# Autodesk Inventor assembly: M178-1000
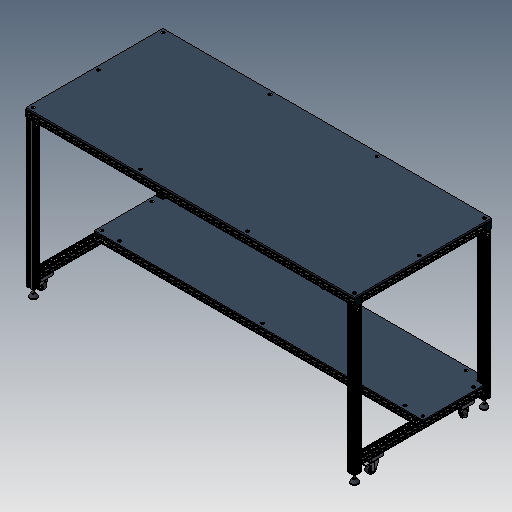
[picture p0: Inventor's stored thumbnail of the model, 512x512]
Saved by Autodesk Inventor 2018.3 (Build 223284000, 284)
## iProperties
Created: 2004-11-17
Part Number: M178-1000
Document SubType Name: Assembly
Designer: Autodesk, Inc.
Manufacturer: Standard
Standards Organization: Custom
Description: TABLE, MAIN
Mass: 47415.2 g
Surface Area: 115729 cm^2
Volume: 28165.1 cm^3
Density: 1.68347 g/cm^3
CAGE: 1LJX3
Dept. ID: Product Design
Description #2: ---
Finish #1: ---
Finish #2: ---
Material ID: ---
Project Number: ---
Author: Autodesk, Inc.
## Documents named in this file (14)
- C:\AVAInvAPI\Workspace\Test Station\Components\M178-1000.iam
- C:\AVAInvAPI\Workspace\Test Station\Components\M178-1001.ipt
- C:\AVAInvAPI\Workspace\Test Station\Components\M178-1007.ipt
- C:\AVAInvAPI\Workspace\Test Station\Components\M178-1005.ipt
- C:\AVAInvAPI\Workspace\Test Station\Components\M178-1100.iam
- C:\AVAInvAPI\Workspace\Test Station\Components\M178-1000-Phantom01.iam
- C:\AVAInvAPI\Workspace\Test Station\Components\M178-1000_Leg_Phantom.iam
- C:\AVAInvAPI\Workspace\Test Station\Components\18-813.ipt
- C:\AVAInvAPI\Workspace\Test Station\Components\20-004.iam
- C:\AVAInvAPI\Workspace\Test Station\Components\M178-100_Cross_Phantom.iam
- C:\AVAInvAPI\Workspace\Test Station\Components\21-092 Caster Phantom.iam
- C:\AVAInvAPI\Workspace\Test Station\Components\21-091 Caster Phantom.iam
- C:\Users\kelleyb.ADS\Desktop\Samples MIGRATED 2009 224 RTM_1\Standard Parts\Test Station Content\Extrusions\40 Series Profiles.ipt
- C:\Users\kelleyb.ADS\Desktop\Samples MIGRATED 2009 224 RTM_1\Standard Parts\Test Station Content\End Caps\18-xxx 40 Series End Caps.ipt
## Components (43 placed, 11 different names)
1. M178-1001:1 — Mate:1, Flush:1, Flush:2, Insert:1
2. M178-1100:1 [sub-assembly] — Mate:1, Flush:1, Flush:2, Mate:2, Flush:3, Flush:4, Insert:8, Insert:9, Insert:10, Insert:11, Angle:5, Angle:6, Angle:7, Angle:8
3. M178-1005:1 — Mate:3, Flush:7, Insert:2, Angle:1, Insert:3, Angle:2, Mate:6, Flush:12, Flush:14, Mate:8, Flush:16, Mate:10, Flush:17, Flush:24
4. M178-1005:2 — Mate:5, Flush:11, Insert:4, Angle:3, Insert:5, Angle:4, Flush:19, Mate:12, Flush:20, Mate:14, Flush:21
5. 20-004:1 [sub-assembly] — Insert:2, Angle:1
6. 20-004:2 [sub-assembly] — Insert:3, Angle:2
7. 20-004:3 [sub-assembly] — Insert:5, Angle:4
8. 20-004:4 [sub-assembly] — Insert:4, Angle:3
9. M178-100_Cross_Phantom:1 [sub-assembly] — Mate:6, Flush:12, Flush:13, Flush:19, Flush:23
10. M178-100_Cross_Phantom:2 [sub-assembly] — Flush:14, Flush:15, Mate:7, Flush:22
11. 21-092 Caster Phantom:1 [sub-assembly] — Mate:10, Flush:17, Mate:11
12. 21-091 Caster Phantom:1 [sub-assembly] — Mate:8, Flush:16, Mate:9, Flush:18
13. 21-092 Caster Phantom:2 [sub-assembly] — Mate:14, Flush:21, Mate:15
14. 21-091 Caster Phantom:2 [sub-assembly] — Mate:12, Flush:20, Mate:13
15. M178-1007:1 — Flush:22, Flush:23, Flush:24, Insert:6, Insert:7
16. 18-813:1 — Insert:8, Angle:8
17. 18-813:2 — Insert:9, Angle:7
18. 18-813:3 — Insert:10, Angle:5
19. 18-813:4 — Insert:11, Angle:6
20. M178-1000-Phantom01:1 [sub-assembly] — Insert:1
21. M178-1000-Phantom01:11 [sub-assembly]
22. M178-1000-Phantom01:3 [sub-assembly]
23. M178-1000-Phantom01:4 [sub-assembly]
24. M178-1000-Phantom01:5 [sub-assembly]
25. M178-1000-Phantom01:6 [sub-assembly]
26. M178-1000-Phantom01:7 [sub-assembly]
27. M178-1000-Phantom01:8 [sub-assembly]
28. M178-1000-Phantom01:12 [sub-assembly]
29. M178-1000-Phantom01:10 [sub-assembly]
30. M178-1000_Leg_Phantom:1 [sub-assembly] — Mate:2, Flush:3, Flush:4, Mate:3, Flush:7, Flush:13, Mate:11, Mate:16
31. M178-1000_Leg_Phantom:2 [sub-assembly] — Flush:15, Mate:7, Mate:9
32. M178-1000_Leg_Phantom:3 [sub-assembly] — Mate:5, Flush:11, Mate:15
33. M178-1000_Leg_Phantom:4 [sub-assembly] — Mate:13
34. M178-1000-Phantom01:13 [sub-assembly] — Insert:6
35. M178-1000-Phantom01:15 [sub-assembly]
36. M178-1000-Phantom01:16 [sub-assembly]
37. M178-1000-Phantom01:17 [sub-assembly]
38. M178-1000-Phantom01:14 [sub-assembly] — Insert:7
39. M178-1000-Phantom01:18 [sub-assembly]
40. M178-1000-Phantom01:19 [sub-assembly]
41. M178-1000-Phantom01:20 [sub-assembly]
42. M178-1000-Phantom01:21 [sub-assembly]
43. M178-1000-Phantom01:22 [sub-assembly]
## Component patterns: (12 elements, first: M178-1000-Phantom01:1), (4 elements, first: M178-1000_Leg_Phantom:1), (4 elements, first: M178-1000-Phantom01:13), (6 elements, first: M178-1000-Phantom01:14)
## Relationships (53: Flush 19, Mate 15, Insert 11, Angle 8)
- Mate:1: M178-1001:1 ↔ M178-1100:1
- Flush:1: M178-1001:1 ↔ M178-1100:1
- Flush:2: M178-1001:1 ↔ M178-1100:1
- Insert:1: M178-1001:1 ↔ M178-1000-Phantom01:1
- Mate:2: M178-1100:1 ↔ M178-1000_Leg_Phantom:1
- Flush:3: M178-1100:1 ↔ M178-1000_Leg_Phantom:1
- Flush:4: M178-1100:1 ↔ M178-1000_Leg_Phantom:1
- Mate:3: M178-1005:1 ↔ M178-1000_Leg_Phantom:1
- Flush:7: M178-1005:1 ↔ M178-1000_Leg_Phantom:1
- Mate:5: M178-1005:2 ↔ M178-1000_Leg_Phantom:3
- Flush:11: M178-1005:2 ↔ M178-1000_Leg_Phantom:3
- Insert:2: M178-1005:1 ↔ 20-004:1
- Angle:1 (0 deg): M178-1005:1 ↔ 20-004:1
- Insert:3: M178-1005:1 ↔ 20-004:2
- Angle:2 (0 deg): M178-1005:1 ↔ 20-004:2
- Insert:4: M178-1005:2 ↔ 20-004:4
- Angle:3 (0 deg): M178-1005:2 ↔ 20-004:4
- Insert:5: M178-1005:2 ↔ 20-004:3
- Angle:4 (0 deg): M178-1005:2 ↔ 20-004:3
- Mate:6: M178-1005:1 ↔ M178-100_Cross_Phantom:1
- Flush:12: M178-1005:1 ↔ M178-100_Cross_Phantom:1
- Flush:13 (381 mm): M178-100_Cross_Phantom:1 ↔ M178-1000_Leg_Phantom:1
- Flush:14: M178-1005:1 ↔ M178-100_Cross_Phantom:2
- Flush:15: M178-100_Cross_Phantom:2 ↔ M178-1000_Leg_Phantom:2
- Mate:7: M178-100_Cross_Phantom:2 ↔ M178-1000_Leg_Phantom:2
- Mate:8: M178-1005:1 ↔ 21-091 Caster Phantom:1
- Flush:16: M178-1005:1 ↔ 21-091 Caster Phantom:1
- Mate:9 (50.8 mm): 21-091 Caster Phantom:1 ↔ M178-1000_Leg_Phantom:2
- Mate:10: M178-1005:1 ↔ 21-092 Caster Phantom:1
- Flush:17: M178-1005:1 ↔ 21-092 Caster Phantom:1
- Mate:11: 21-092 Caster Phantom:1 ↔ M178-1000_Leg_Phantom:1
- Flush:18: 21-091 Caster Phantom:1
- Flush:19: M178-1005:2 ↔ M178-100_Cross_Phantom:1
- Mate:12: M178-1005:2 ↔ 21-091 Caster Phantom:2
- Flush:20: M178-1005:2 ↔ 21-091 Caster Phantom:2
- Mate:13 (50.8 mm): 21-091 Caster Phantom:2 ↔ M178-1000_Leg_Phantom:4
- Mate:14: M178-1005:2 ↔ 21-092 Caster Phantom:2
- Flush:21: M178-1005:2 ↔ 21-092 Caster Phantom:2
- Mate:15 (50.8 mm): 21-092 Caster Phantom:2 ↔ M178-1000_Leg_Phantom:3
- Flush:22: M178-100_Cross_Phantom:2 ↔ M178-1007:1
- Flush:23: M178-100_Cross_Phantom:1 ↔ M178-1007:1
- Flush:24: M178-1005:1 ↔ M178-1007:1
- Insert:6: M178-1007:1 ↔ M178-1000-Phantom01:13
- Insert:7: M178-1007:1 ↔ M178-1000-Phantom01:14
- Mate:16: M178-1000_Leg_Phantom:1
- Insert:8: M178-1100:1 ↔ 18-813:1
- Insert:9: M178-1100:1 ↔ 18-813:2
- Insert:10: M178-1100:1 ↔ 18-813:3
- Insert:11: M178-1100:1 ↔ 18-813:4
- Angle:5 (0 deg): M178-1100:1 ↔ 18-813:3
- Angle:6 (0 deg): M178-1100:1 ↔ 18-813:4
- Angle:7 (0 deg): M178-1100:1 ↔ 18-813:2
- Angle:8 (0 deg): M178-1100:1 ↔ 18-813:1
